# Autodesk Inventor assembly: !Ramp
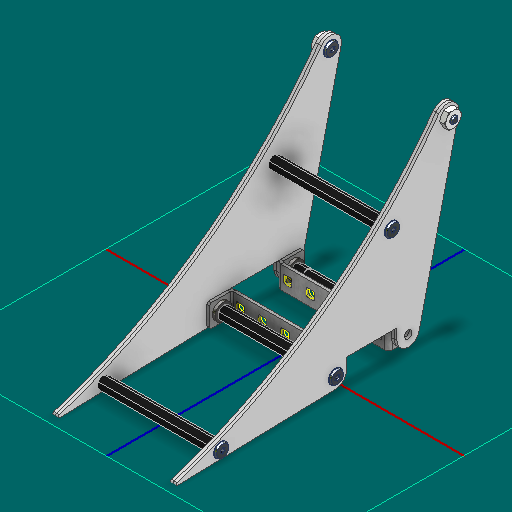
[picture p0: Inventor's stored thumbnail of the model, 512x512]
Saved by Autodesk Inventor 2025 (Build 290162000, 162)
## iProperties
Created: 2024-10-21
Part Number: !Ramp
Document SubType Name: Assembly
Designer: averey
Author: averey
## Documents named in this file (15)
- C:\Users\avere\VEX\High Stakes\CAD\V2\Intake\Ramp\!Ramp.iam
- C:\Users\avere\VEX\High Stakes\CAD\ROBOPROS-CAD-Inventor\Structure\C Channel\Aluminum 1x5x1\Alu C 1x5x1x1.ipt
- C:\Users\avere\VEX\High Stakes\CAD\V2\Intake\Custom Parts\Ramp.ipt
- C:\Users\avere\VEX\High Stakes\CAD\ROBOPROS-CAD-Inventor\Structure\Standoff\Standoff 2.50.ipt
- C:\Users\avere\VEX\High Stakes\CAD\ROBOPROS-CAD-Inventor\Structure\Standoff.ipt
- C:\Users\avere\VEX\High Stakes\CAD\ROBOPROS-CAD-Inventor\Structure\Hardware\Screw Steel - Star\SScrew Star Smooth .290.ipt
- C:\Users\avere\VEX\High Stakes\CAD\ROBOPROS-CAD-Inventor\Structure\Hardware\Screw Steel - Star.ipt
- C:\Users\avere\VEX\High Stakes\CAD\ROBOPROS-CAD-Inventor\Structure\Hardware\Screw Shoulder Robosource\SScrew Shoulder Smooth .500 x .18.ipt
- C:\Users\avere\VEX\High Stakes\CAD\ROBOPROS-CAD-Inventor\Structure\Hardware\Screw Shoulder Robosource.ipt
- C:\Users\avere\VEX\High Stakes\CAD\ROBOPROS-CAD-Inventor\Structure\Standoff\Standoff .25.ipt
- C:\Users\avere\VEX\High Stakes\CAD\ROBOPROS-CAD-Inventor\Structure\Standoff\Standoff 2.00.ipt
- C:\Users\avere\VEX\High Stakes\CAD\ROBOPROS-CAD-Inventor\Motion\Spacers\Washer Steel\SWasher .375 OD x .062500.ipt
- C:\Users\avere\VEX\High Stakes\CAD\ROBOPROS-CAD-Inventor\Motion\Spacers\Washer Steel.ipt
- C:\Users\avere\VEX\High Stakes\CAD\ROBOPROS-CAD-Inventor\Structure\Hardware\Nut Nylon\Nut Nylon - White.ipt
- C:\Users\avere\VEX\High Stakes\CAD\ROBOPROS-CAD-Inventor\Structure\Hardware\Nut Nylon.ipt
## Components (25 placed, 9 different names)
1. Alu C 1x5x1x1:1 — Mate:3, Mate:4, Mate:5, Mate:6, Mate:7, Angle:1, Insert:4, Insert:13, Insert:14, Insert:15
2. Alu C 1x5x1x1:2 — Mate:3, Mate:4, Mate:8, Mate:9, Mate:11, Insert:17
3. Ramp:1 — Insert:7, Insert:8, Insert:11, Insert:21
4. Ramp:2 — Insert:20
5. Ramp:3 — Insert:4, Mate:11, Insert:5, Insert:6, Insert:22
6. Ramp:4 — Insert:9, Insert:10, Insert:23
7. Standoff 2.50:1 — Insert:5
8. Standoff 2.50:2 — Insert:6
9. SScrew Star Smooth .290:1 — Insert:8
10. SScrew Star Smooth .290:2 — Insert:7
11. SScrew Star Smooth .290:3 — Insert:9
12. SScrew Shoulder Smooth .500 x .18:1 — Insert:10
13. SScrew Shoulder Smooth .500 x .18:2 — Insert:11
14. Standoff .25:3 — Insert:12, Insert:13
15. Standoff 2.00:4 — Insert:12
16. SWasher .375 OD x .062500:1 — Insert:14
17. SWasher .375 OD x .062500:2 — Insert:15
18. Standoff .25:5 — Insert:19
19. Standoff 2.00:6 — Insert:18
20. SWasher .375 OD x .062500:3 — Insert:17, Insert:18
21. SWasher .375 OD x .062500:4 — Insert:19
22. SScrew Star Smooth .290:4 — Insert:20
23. Nut Nylon - White:1 — Insert:21
24. SScrew Star Smooth .290:5 — Insert:22
25. Nut Nylon - White:2 — Insert:23
## Relationships (35: Insert 23, Mate 11, Angle 1)
- [Insert]: Ramp:1 ↔ Ramp:2
- [Mate]: Ramp:1 ↔ Ramp:2
- [Insert]: Alu C 1x5x1x1:1 ↔ Ramp:2
- [Mate]: Alu C 1x5x1x1:2 ↔ Ramp:1
- Mate:3: Alu C 1x5x1x1:1 ↔ Alu C 1x5x1x1:2
- Mate:4: Alu C 1x5x1x1:1 ↔ Alu C 1x5x1x1:2
- Mate:5: Alu C 1x5x1x1:1
- Mate:6: Alu C 1x5x1x1:1
- Mate:7: Alu C 1x5x1x1:1
- Mate:8: Alu C 1x5x1x1:2
- Mate:9: Alu C 1x5x1x1:2
- Angle:1 (0 deg): Alu C 1x5x1x1:1
- [Insert]: Ramp:3 ↔ Ramp:4
- [Mate]: Ramp:3 ↔ Ramp:4
- Insert:4: Alu C 1x5x1x1:1 ↔ Ramp:3
- Mate:11: Alu C 1x5x1x1:2 ↔ Ramp:3
- Insert:5: Ramp:3 ↔ Standoff 2.50:1
- Insert:6: Ramp:3 ↔ Standoff 2.50:2
- Insert:7: Ramp:1 ↔ SScrew Star Smooth .290:2
- Insert:8: Ramp:1 ↔ SScrew Star Smooth .290:1
- Insert:9: Ramp:4 ↔ SScrew Star Smooth .290:3
- Insert:10: Ramp:4 ↔ SScrew Shoulder Smooth .500 x .18:1
- Insert:11: Ramp:1 ↔ SScrew Shoulder Smooth .500 x .18:2
- Insert:12: Standoff .25:3 ↔ Standoff 2.00:4
- Insert:13 (1.5875 mm): Alu C 1x5x1x1:1 ↔ Standoff .25:3
- Insert:14: Alu C 1x5x1x1:1 ↔ SWasher .375 OD x .062500:1
- Insert:15: Alu C 1x5x1x1:1 ↔ SWasher .375 OD x .062500:2
- [Insert]: Standoff .25:5 ↔ Standoff 2.00:6
- Insert:17: Alu C 1x5x1x1:2 ↔ SWasher .375 OD x .062500:3
- Insert:18: Standoff 2.00:6 ↔ SWasher .375 OD x .062500:3
- Insert:19: Standoff .25:5 ↔ SWasher .375 OD x .062500:4
- Insert:20: Ramp:2 ↔ SScrew Star Smooth .290:4
- Insert:21: Ramp:1 ↔ Nut Nylon - White:1
- Insert:22: Ramp:3 ↔ SScrew Star Smooth .290:5
- Insert:23: Ramp:4 ↔ Nut Nylon - White:2
## Named parameters: d12_d48 = 0 mm, d13_d49 = 0 mm, d28_d24 = 0 mm
